# Autodesk Inventor assembly: 317-03
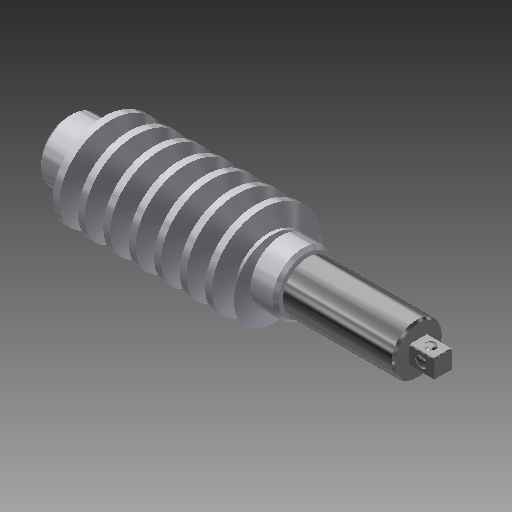
[picture p0: Inventor's stored thumbnail of the model, 512x512]
Saved by Autodesk Inventor 2019 (Build 230136000, 136)
## iProperties
Company: Autodesk Inc.
Created: 2008-01-21
Part Number: 317-03
Document SubType Name: Assembly
Designer: Autodesk Inc.
Mass: 13.5221 g
Surface Area: 38.9294 cm^2
Volume: 5.08535 cm^3
Density: 2.65902 g/cm^3
Author: Inventor
## Documents named in this file (3)
- C:\TEMP\Car Seat\Workspace\Rear Worm Motor Shaft.iam
- C:\TEMP\Car Seat\Workspace\Motor Shaft.ipt
- C:\TEMP\Car Seat\Workspace\Worm Gear.ipt
## Components (2 placed, 2 different names)
1. Motor Shaft:1 — Insert:1
2. Worm:1 — Insert:1
## Relationships (1: Insert 1)
- Insert:1: Motor Shaft:1 ↔ Worm:1
